# Autodesk Inventor assembly: Multi_Op_Setup_Flats
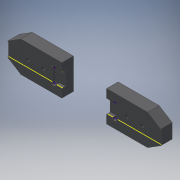
[picture p0: Inventor's stored thumbnail of the model, 180x180]
Saved by Autodesk Inventor 2018.3 (Build 223284000, 284)
## iProperties
Created: 2018-12-07
Part Number: Multi_Op_Setup_Flats
Project: =<Part Number>
Document SubType Name: Assembly
Designer: machinetools
Author: machinetools
## Documents named in this file (2)
- R:\CAD\~Aquafil~\7407 - 456 Slant Blades-72 Flat Blades (Standard Size)\CAD\Multi_Op_Setup_Flats.iam
- R:\CAD\~Aquafil~\7407 - 456 Slant Blades-72 Flat Blades (Standard Size)\CAD\DHC-1500-FF-02-002.ipt
## Components (2 placed, 1 different names)
1. DHC-1500-FF-02-002:1 — Flush:1, Flush:2, Mate:1
2. DHC-1500-FF-02-002:2 — Flush:1, Flush:2, Mate:1
## Relationships (3: Flush 2, Mate 1)
- Flush:1: DHC-1500-FF-02-002:1 ↔ DHC-1500-FF-02-002:2
- Flush:2: DHC-1500-FF-02-002:1 ↔ DHC-1500-FF-02-002:2
- Mate:1 (-397.4846 mm): DHC-1500-FF-02-002:1 ↔ DHC-1500-FF-02-002:2
